# Autodesk Inventor assembly: PI holder_2p0
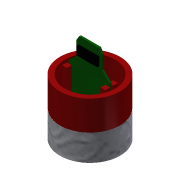
[picture p0: Inventor's stored thumbnail of the model, 180x180]
Saved by Autodesk Inventor 2014 (Build 180170000, 170)
## iProperties
Created: 2016-10-07
Part Number: PI holder_2p0
Document SubType Name: Assembly
Designer: Camilo
Author: Camilo
## Documents named in this file (4)
- Z:\Github\AgingTests\3D parts\PI holder_2p0\PI holder_2p0.iam
- Z:\Github\AgingTests\3D parts\PI holder_2p0\bottleCap.ipt
- Z:\Github\AgingTests\3D parts\PI holder_2p0\PI_holder.ipt
- Z:\Github\AgingTests\3D parts\PI holder\WirebondAdapter.ipt
## Components (3 placed, 3 different names)
1. bottleCap:1 — Flush:1
2. PI_holder:1 — Flush:1, Mate:2
3. WirebondAdapter:1 — Mate:1, Mate:2, Flush:2
## Relationships (4: Flush 2, Mate 2)
- Flush:1: bottleCap:1 ↔ PI_holder:1
- Mate:1 (0.38 mm): WirebondAdapter:1
- Mate:2: PI_holder:1 ↔ WirebondAdapter:1
- Flush:2: WirebondAdapter:1
